# Autodesk Inventor assembly: Robot_assembly
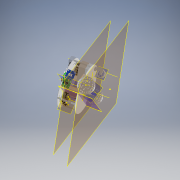
[picture p0: Inventor's stored thumbnail of the model, 180x180]
Saved by Autodesk Inventor 2020 (Build 240168000, 168)
## iProperties
Created: 2020-07-10
Part Number: Robot_assembly
Document SubType Name: Assembly
Designer: Sičaja
Author: Sičaja
## Documents named in this file (13)
- C:\Users\Sicaja\Documents\Draws_Inventor\Inventor_Robocup\Robot_assembly.iam
- C:\Users\Sicaja\Documents\Draws_Inventor\Inventor_Robocup\KonstrukcijaDonjiDio_v.1.2.ipt
- C:\Users\Sicaja\Documents\Draws_Inventor\Inventor_Robocup\Kotač_konekcija_v.1.0.ipt
- C:\Users\Sicaja\Documents\Draws_Inventor\Inventor_Robocup\Kotač_v.2.0.ipt
- C:\Users\Sicaja\Documents\Draws_Inventor\Inventor_Robocup\GornjaKonstrukcija_v.1.1.iam
- C:\Users\Sicaja\Documents\Draws_Inventor\Inventor_Robocup\mrm-lid-an.ipt
- C:\Users\Sicaja\Documents\Draws_Inventor\Inventor_Robocup\Raspberry Pi 4 Model B\Raspberry Pi 4 Model B.iam
- C:\Users\Sicaja\Documents\Draws_Inventor\Inventor_Robocup\Raspberry Pi Camera Module 2.1\Cam V2.1 v1.ipt
- C:\Users\Sicaja\Documents\Draws_Inventor\Inventor_Robocup\AdfruitThermalSensor\Camara AMG8833.ipt
- C:\Users\Sicaja\Documents\Draws_Inventor\Inventor_Robocup\KonstrukcijaDonjiDio_v.1.2_MIR.ipt
- C:\Users\Sicaja\Documents\Draws_Inventor\Inventor_Robocup\AdfruitThermalSensor\Camara AMG8833_MIR.ipt
- C:\Users\Sicaja\Documents\Draws_Inventor\Inventor_Robocup\Raspberry Pi Camera Module 2.1\Cam V2.1 v1_MIR.ipt
- C:\Users\Sicaja\Documents\Draws_Inventor\Inventor_Robocup\PrednjiKotač_v.1.0.ipt
## Components (16 placed, 12 different names)
1. KonstrukcijaDonjiDio_v.1.2:1 — Mate:1, Insert:1, Insert:3, Flush:1, Mate:2, Mate:3, Mate:4, Angle:1, Insert:23, Insert:24, Mate:15
2. Kotač_konekcija_v.1.0:1 — Mate:1, Insert:1, Insert:2
3. Kotač_v.2.0:1 — Insert:2, Symmetry:1, Tangent:1
4. Kotač_v.2.0:2 — Insert:4, Symmetry:1
5. Kotač_konekcija_v.1.0:2 — Insert:3, Insert:4
6. GornjaKonstrukcija_v.1.1:1 [sub-assembly] — Mate:2, Mate:3, Mate:4, Insert:7, Insert:8, Mate:9, Mate:10, Mate:11, Mate:12, Mate:13, Mate:14, Insert:17, Insert:18, Insert:19, Insert:20, Insert:21, Insert:22
7. Raspberry Pi 4 Model B:1 [sub-assembly] — Insert:7, Insert:8
8. Camara AMG8833:2 — Mate:12, Mate:13, Mate:14
9. Cam V2.1 v1:3 — Mate:9, Mate:10, Mate:11
10. KonstrukcijaDonjiDio_v.1.2_MIR:1
11. Camara AMG8833_MIR:1
12. Cam V2.1 v1_MIR:1
13. mrm-lid-an:6 — Insert:19, Insert:20
14. mrm-lid-an:8 — Insert:21, Insert:22
15. mrm-lid-an:10 — Insert:17, Insert:18
16. PrednjiKotač_v.1.0:1 — Insert:23, Insert:24, Mate:15
## Relationships (30: Insert 14, Mate 11, Flush 2, Symmetry 1, Angle 1, Tangent 1)
- Mate:1: KonstrukcijaDonjiDio_v.1.2:1 ↔ Kotač_konekcija_v.1.0:1
- Insert:1: KonstrukcijaDonjiDio_v.1.2:1 ↔ Kotač_konekcija_v.1.0:1
- Insert:2: Kotač_konekcija_v.1.0:1 ↔ Kotač_v.2.0:1
- Insert:3: KonstrukcijaDonjiDio_v.1.2:1 ↔ Kotač_konekcija_v.1.0:2
- Insert:4: Kotač_v.2.0:2 ↔ Kotač_konekcija_v.1.0:2
- Flush:1 (-31.434 mm): KonstrukcijaDonjiDio_v.1.2:1
- Symmetry:1: Kotač_v.2.0:1 ↔ Kotač_v.2.0:2
- Mate:2: KonstrukcijaDonjiDio_v.1.2:1 ↔ GornjaKonstrukcija_v.1.1:1
- Mate:3: KonstrukcijaDonjiDio_v.1.2:1 ↔ GornjaKonstrukcija_v.1.1:1
- Mate:4: KonstrukcijaDonjiDio_v.1.2:1 ↔ GornjaKonstrukcija_v.1.1:1
- Insert:7: GornjaKonstrukcija_v.1.1:1 ↔ Raspberry Pi 4 Model B:1
- Insert:8: GornjaKonstrukcija_v.1.1:1 ↔ Raspberry Pi 4 Model B:1
- Mate:9: GornjaKonstrukcija_v.1.1:1 ↔ Cam V2.1 v1:3
- Mate:10: GornjaKonstrukcija_v.1.1:1 ↔ Cam V2.1 v1:3
- Mate:11 (-1 mm): GornjaKonstrukcija_v.1.1:1 ↔ Cam V2.1 v1:3
- Mate:12: GornjaKonstrukcija_v.1.1:1 ↔ Camara AMG8833:2
- Mate:13 (-1 mm): GornjaKonstrukcija_v.1.1:1 ↔ Camara AMG8833:2
- Mate:14: GornjaKonstrukcija_v.1.1:1 ↔ Camara AMG8833:2
- Insert:17: GornjaKonstrukcija_v.1.1:1 ↔ mrm-lid-an:10
- Insert:18: GornjaKonstrukcija_v.1.1:1 ↔ mrm-lid-an:10
- Insert:19: GornjaKonstrukcija_v.1.1:1 ↔ mrm-lid-an:6
- Insert:20: GornjaKonstrukcija_v.1.1:1 ↔ mrm-lid-an:6
- Insert:21: GornjaKonstrukcija_v.1.1:1 ↔ mrm-lid-an:8
- Insert:22: GornjaKonstrukcija_v.1.1:1 ↔ mrm-lid-an:8
- Angle:1 (0 deg): KonstrukcijaDonjiDio_v.1.2:1
- Tangent:1: Kotač_v.2.0:1
- Flush:2 (50 mm)
- Insert:23: KonstrukcijaDonjiDio_v.1.2:1 ↔ PrednjiKotač_v.1.0:1
- Insert:24: KonstrukcijaDonjiDio_v.1.2:1 ↔ PrednjiKotač_v.1.0:1
- Mate:15: KonstrukcijaDonjiDio_v.1.2:1 ↔ PrednjiKotač_v.1.0:1
